# Autodesk Inventor assembly: scrambler_assy1
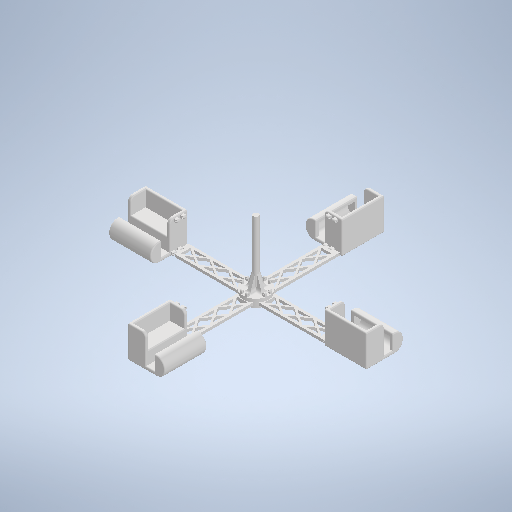
[picture p0: Inventor's stored thumbnail of the model, 512x512]
Saved by Autodesk Inventor 2025.2 (Build 292293000, 293)
## iProperties
Created: 2025-10-10
Part Number: scrambler_assy1
Document SubType Name: Assembly
Designer: pascu
Author: pascu
## Documents named in this file (4)
- C:\Users\pascu\OneDrive\Documents\GitHub\amusement-park\scrambler_assy1.iam
- C:\Users\pascu\OneDrive\Documents\GitHub\amusement-park\scrambler_chariot.ipt
- C:\Users\pascu\OneDrive\Documents\GitHub\amusement-park\scrambler_spider_beam.ipt
- C:\Users\pascu\OneDrive\Documents\GitHub\amusement-park\scrambler_vertical_outer.ipt
## Components (9 placed, 3 different names)
1. scrambler_chariot:1 — Mate:1, Angle:1, Flush:1
2. scrambler_spider_beam:1 — Mate:1, Angle:1, Flush:1, Mate:2, Mate:3
3. scrambler_vertical_outer:1 — Mate:2, Mate:3, Mate:8, Mate:9, Mate:10, Mate:11, Mate:12, Mate:13
4. scrambler_chariot:2
5. scrambler_spider_beam:2 — Mate:8, Mate:9
6. scrambler_chariot:3
7. scrambler_spider_beam:3 — Mate:12, Mate:13
8. scrambler_chariot:4
9. scrambler_spider_beam:4 — Mate:10, Mate:11
## Relationships (20: Mate 12, Angle 4, Flush 4)
- Mate:1: scrambler_chariot:1 ↔ scrambler_spider_beam:1
- Angle:1 (0 deg): scrambler_chariot:1 ↔ scrambler_spider_beam:1
- Flush:1 (-11.43 mm): scrambler_chariot:1 ↔ scrambler_spider_beam:1
- Mate:2: scrambler_spider_beam:1 ↔ scrambler_vertical_outer:1
- Mate:3: scrambler_spider_beam:1 ↔ scrambler_vertical_outer:1
- [Mate]: scrambler_chariot:2 ↔ scrambler_spider_beam:2
- [Angle] (0 deg): scrambler_chariot:2 ↔ scrambler_spider_beam:2
- [Flush] (-11.43 mm): scrambler_chariot:2 ↔ scrambler_spider_beam:2
- [Mate]: scrambler_chariot:3 ↔ scrambler_spider_beam:3
- [Angle] (0 deg): scrambler_chariot:3 ↔ scrambler_spider_beam:3
- [Flush] (-11.43 mm): scrambler_chariot:3 ↔ scrambler_spider_beam:3
- [Mate]: scrambler_chariot:4 ↔ scrambler_spider_beam:4
- [Angle] (0 deg): scrambler_chariot:4 ↔ scrambler_spider_beam:4
- [Flush] (-11.43 mm): scrambler_chariot:4 ↔ scrambler_spider_beam:4
- Mate:8: scrambler_vertical_outer:1 ↔ scrambler_spider_beam:2
- Mate:9: scrambler_vertical_outer:1 ↔ scrambler_spider_beam:2
- Mate:10: scrambler_vertical_outer:1 ↔ scrambler_spider_beam:4
- Mate:11: scrambler_vertical_outer:1 ↔ scrambler_spider_beam:4
- Mate:12: scrambler_vertical_outer:1 ↔ scrambler_spider_beam:3
- Mate:13: scrambler_vertical_outer:1 ↔ scrambler_spider_beam:3
## Named parameters: d7_d1 = 0 mm, d8_d2 = 0 deg, d9_d3 = -11.43 mm, d10_d1 = 0 mm, d11_d2 = 0 deg, d12_d3 = -11.43 mm, d13_d1 = 0 mm, d14_d2 = 0 deg, d15_d3 = -11.43 mm
